# Autodesk Inventor assembly: climber assembly
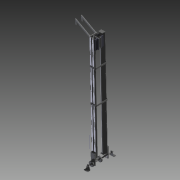
[picture p0: Inventor's stored thumbnail of the model, 180x180]
Saved by Autodesk Inventor 2013 (Build 170138000, 138)
## iProperties
Created: 2013-01-19
Part Number: climber assembly
Document SubType Name: Assembly
Designer: Arpan
Author: Arpan
## Documents named in this file (13)
- C:\Users\Arpan\Documents\GitHub\frc2013CAD\Climber\climber assembly.iam
- C:\Users\Arpan\Documents\GitHub\frc2013CAD\Climber\Slide rale 39.5.ipt
- C:\Users\Arpan\Documents\GitHub\frc2013CAD\Climber\Linear bearing.ipt
- C:\Users\Arpan\Documents\GitHub\frc2013CAD\Climber\bearing faceplate.ipt
- C:\Users\Arpan\Documents\GitHub\frc2013CAD\Climber\endstop.ipt
- C:\Users\Arpan\Documents\GitHub\frc2013CAD\Climber\Generic brace.ipt
- C:\Users\Arpan\Documents\GitHub\frc2013CAD\Climber\arm mount.ipt
- C:\Users\Arpan\Documents\GitHub\frc2013CAD\Climber\bearing 3 8 id 1-1 8 od.ipt
- C:\Users\Arpan\Documents\GitHub\frc2013CAD\Climber\Shaft.ipt
- C:\Users\Arpan\Documents\GitHub\frc2013CAD\Climber\rough pulley.ipt
- C:\Users\Arpan\Documents\GitHub\frc2013CAD\Climber\arm assembly mount plate.ipt
- C:\Users\Arpan\Documents\GitHub\frc2013CAD\Climber\hook mount plate.ipt
- C:\Users\Arpan\Documents\GitHub\frc2013CAD\Climber\hook.ipt
## Components (23 placed, 12 different names)
1. Slide rale 39.5:1 — Mate:2, Angle:2, Flush:1, Mate:8, Mate:9, Mate:10, Mate:12, Mate:14, Mate:15, Mate:22, Mate:23, Mate:24
2. Slide rale 39.5:2 — Mate:1, Angle:1, Flush:1, Mate:11, Mate:13, Mate:16, Mate:17, Mate:18, Mate:19, Mate:20, Mate:21, Angle:4
3. Linear bearing:1 — Mate:1, Angle:1, Mate:3, Flush:2, Flush:3, Mate:4, Mate:5
4. Linear bearing:2 — Mate:2, Angle:2, Mate:3, Flush:2, Flush:3, Mate:7, Flush:4, Flush:5, Flush:6
5. bearing faceplate:1 — Mate:4, Mate:5, Mate:42, Flush:10, Flush:11
6. bearing faceplate:2 — Mate:7, Flush:4, Flush:5, Flush:6
7. endstop:2 — Mate:8, Mate:9, Angle:4
8. Generic brace:2 — Mate:14, Mate:15, Mate:16, Mate:17, Mate:18
9. Generic brace:3 — Mate:10, Mate:11, Mate:12, Mate:13
10. endstop:3 — Mate:19, Mate:20, Mate:21, Mate:25, Mate:26, Mate:27
11. endstop:4 — Mate:22, Mate:23, Mate:24, Mate:28, Mate:29, Mate:30
12. arm mount:1 — Mate:25, Mate:26, Mate:27, Mate:32, Mate:34, Mate:39
13. arm mount:2 — Mate:28, Mate:29, Mate:30, Mate:31, Mate:33, Mate:37, Flush:7, Flush:14, Angle:5
14. bearing 3 8 id 1-1 8 od:1 — Mate:31, Mate:33
15. bearing 3 8 id 1-1 8 od:2 — Mate:32, Mate:34, Mate:35
16. Shaft:1 — Mate:35, Mate:36, Mate:38, Flush:7, Mate:40, Mate:41, Flush:8, Flush:9
17. rough pulley:1 — Mate:36, Mate:37
18. rough pulley:2 — Mate:38, Mate:39
19. arm assembly mount plate:1 — Mate:40, Flush:9, Angle:5
20. arm assembly mount plate:2 — Mate:41, Flush:8
21. hook mount plate:1 — Mate:42, Flush:10, Flush:11, Mate:43, Mate:44, Flush:12, Flush:13, Mate:48, Mate:49
22. hook:1 — Mate:44, Flush:13, Mate:49
23. hook:2 — Mate:43, Flush:12, Mate:48
## Relationships (63: Mate 45, Flush 14, Angle 4)
- Mate:1: Slide rale 39.5:2 ↔ Linear bearing:1
- Angle:1 (0 deg): Slide rale 39.5:2 ↔ Linear bearing:1
- Mate:2: Slide rale 39.5:1 ↔ Linear bearing:2
- Angle:2 (0 deg): Slide rale 39.5:1 ↔ Linear bearing:2
- Mate:3 (22.2504 mm): Linear bearing:1 ↔ Linear bearing:2
- Flush:1: Slide rale 39.5:1 ↔ Slide rale 39.5:2
- Flush:2: Linear bearing:1 ↔ Linear bearing:2
- Flush:3: Linear bearing:1 ↔ Linear bearing:2
- Mate:4: Linear bearing:1 ↔ bearing faceplate:1
- Mate:5: Linear bearing:1 ↔ bearing faceplate:1
- Mate:7: Linear bearing:2 ↔ bearing faceplate:2
- Flush:4: Linear bearing:2 ↔ bearing faceplate:2
- Flush:5: Linear bearing:2 ↔ bearing faceplate:2
- Flush:6: Linear bearing:2 ↔ bearing faceplate:2
- Mate:8: Slide rale 39.5:1 ↔ endstop:2
- Mate:9: Slide rale 39.5:1 ↔ endstop:2
- Mate:10: Slide rale 39.5:1 ↔ Generic brace:3
- Mate:11: Slide rale 39.5:2 ↔ Generic brace:3
- Mate:12: Slide rale 39.5:1 ↔ Generic brace:3
- Mate:13: Slide rale 39.5:2 ↔ Generic brace:3
- Mate:14: Slide rale 39.5:1 ↔ Generic brace:2
- Mate:15: Slide rale 39.5:1 ↔ Generic brace:2
- Mate:16: Slide rale 39.5:2 ↔ Generic brace:2
- Mate:17: Slide rale 39.5:2 ↔ Generic brace:2
- Mate:18: Slide rale 39.5:2 ↔ Generic brace:2
- Mate:19: Slide rale 39.5:2 ↔ endstop:3
- Mate:20: Slide rale 39.5:2 ↔ endstop:3
- Mate:21: Slide rale 39.5:2 ↔ endstop:3
- Mate:22: Slide rale 39.5:1 ↔ endstop:4
- Mate:23: Slide rale 39.5:1 ↔ endstop:4
- Mate:24: Slide rale 39.5:1 ↔ endstop:4
- Mate:25: endstop:3 ↔ arm mount:1
- Mate:26: endstop:3 ↔ arm mount:1
- Mate:27: endstop:3 ↔ arm mount:1
- Mate:28: endstop:4 ↔ arm mount:2
- Mate:29: endstop:4 ↔ arm mount:2
- Mate:30: endstop:4 ↔ arm mount:2
- Mate:31: arm mount:2 ↔ bearing 3 8 id 1-1 8 od:1
- Mate:32: arm mount:1 ↔ bearing 3 8 id 1-1 8 od:2
- Mate:33: arm mount:2 ↔ bearing 3 8 id 1-1 8 od:1
- Mate:34: arm mount:1 ↔ bearing 3 8 id 1-1 8 od:2
- Mate:35: bearing 3 8 id 1-1 8 od:2 ↔ Shaft:1
- Mate:36: Shaft:1 ↔ rough pulley:1
- Mate:37 (53.7337 mm): arm mount:2 ↔ rough pulley:1
- Mate:38: Shaft:1 ↔ rough pulley:2
- Mate:39 (6.35 mm): arm mount:1 ↔ rough pulley:2
- Flush:7 (60.5663 mm): arm mount:2 ↔ Shaft:1
- Mate:40: Shaft:1 ↔ arm assembly mount plate:1
- Mate:41: Shaft:1 ↔ arm assembly mount plate:2
- Flush:8 (12.7 mm): Shaft:1 ↔ arm assembly mount plate:2
- Flush:9 (12.7 mm): Shaft:1 ↔ arm assembly mount plate:1
- Angle:4 (0 deg): Slide rale 39.5:2 ↔ endstop:2
- Mate:42: bearing faceplate:1 ↔ hook mount plate:1
- Flush:10: bearing faceplate:1 ↔ hook mount plate:1
- Flush:11 (-26.9748 mm): bearing faceplate:1 ↔ hook mount plate:1
- Mate:43: hook mount plate:1 ↔ hook:2
- Mate:44: hook mount plate:1 ↔ hook:1
- Flush:12 (6.35 mm): hook mount plate:1 ↔ hook:2
- Flush:13 (6.35 mm): hook mount plate:1 ↔ hook:1
- Mate:48: hook mount plate:1 ↔ hook:2
- Mate:49: hook mount plate:1 ↔ hook:1
- Flush:14 (139.7 mm): arm mount:2
- Angle:5 (0 deg): arm mount:2 ↔ arm assembly mount plate:1
